# Autodesk Inventor assembly: assem_linact_standalone_newfinger_v2_test
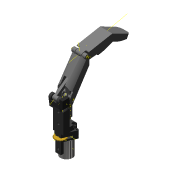
[picture p0: Inventor's stored thumbnail of the model, 180x180]
Saved by Autodesk Inventor 2014 (Build 180170000, 170)
## iProperties
Created: 2015-05-04
Part Number: assem_linact_standalone_newfinger_v2_test
Document SubType Name: Assembly
Designer: Martin
Author: Martin
## Documents named in this file (18)
- C:\Users\Martin\Dropbox\biohand-mec\biohand_v1\fingers\middle\assem_finger_middle.iam
- C:\Users\Martin\Dropbox\biohand-mec\biohand_v1\fingers\index\linact_knuckle_v2.ipt
- C:\Users\Martin\Dropbox\biohand-mec\biohand_v1\fingers\index\assem_linact_rod_v3.iam
- C:\Users\Martin\Dropbox\biohand-mec\biohand_v1\fingers\middle\finger_proximal_v2.ipt
- C:\Users\Martin\Dropbox\biohand-mec\biohand_v1\fingers\index\finger_clevislink.ipt
- C:\Users\Martin\Dropbox\biohand-mec\biohand_v1\misc\servo_square_pot.ipt
- C:\Users\Martin\Dropbox\biohand-mec\biohand_v1\fingers\middle\finger_link_v2.ipt
- C:\Users\Martin\Dropbox\biohand-mec\biohand_v1\fingers\middle\finger_distal.ipt
- C:\Users\Martin\Dropbox\biohand-mec\biohand_v1\misc\bearing_10_4_3.ipt
- C:\Users\Martin\Dropbox\biohand-mec\biohand_v1\misc\m3_25_screw.ipt
- C:\Users\Martin\Dropbox\biohand-mec\biohand_v1\misc\m3_nut.ipt
- C:\Users\Martin\Dropbox\biohand-mec\biohand_v1\misc\servo_gear_2.ipt
- C:\Users\Martin\Dropbox\biohand-mec\biohand_v1\fingers\index\linact_top.ipt
- C:\Users\Martin\Dropbox\biohand-mec\biohand_v1\fingers\index\linact_base.ipt
- C:\Users\Martin\Dropbox\biohand-mec\biohand_v1\misc\m2_8_screw.ipt
- C:\Users\Martin\Dropbox\biohand-mec\biohand_v1\misc\motor_servo.ipt
- C:\Users\Martin\Dropbox\biohand-mec\biohand_v1\misc\m2_4_screw.ipt
- C:\Users\Martin\Dropbox\biohand-mec\biohand_v1\misc\servo_gear_1.ipt
## Components (23 placed, 17 different names)
1. linact_knuckle_v2:1 — Mate:1, Mate:2, Insert:1, Insert:3, Insert:4, Insert:6, Mate:6, Mate:7, Mate:8, Insert:12
2. assem_linact_rod_v3:1 [sub-assembly] — Mate:1, Mate:2, Insert:2
3. finger_proximal_v2:1 — Insert:1, Mate:3, Insert:5, Angle:2, Insert:9, Insert:14, Insert:15, Insert:16, Insert:17, Insert:18, Insert:19
4. finger_clevislink:1 — Insert:2, Mate:3
5. servo_square_pot:1 — Insert:3, Angle:1
6. finger_link_v2:1 — Insert:4, Mate:4, Insert:10
7. finger_distal:1 — Insert:5, Mate:4, Insert:9
8. bearing_10_4_3:1 — Insert:6, Insert:8
9. m3_25_screw:1 — Insert:7
10. m3_nut:1 — Mate:5, Insert:8
11. servo_gear_2:1 — Mate:5, Insert:7
12. linact_top:1 — Mate:6, Mate:7, Mate:8, Mate:9, Mate:10, Mate:11, Insert:13
13. linact_base:1 — Mate:9, Mate:10, Mate:11, Insert:11
14. m2_8_screw:1 — Insert:10
15. motor_servo:1 — Insert:11, Angle:3
16. m2_4_screw:1 — Insert:12
17. servo_gear_1:1 — Insert:13
18. m2_8_screw:2 — Insert:14
19. m2_8_screw:3 — Insert:15
20. m2_8_screw:4 — Insert:18
21. m2_8_screw:5 — Insert:16
22. m2_8_screw:6 — Insert:17
23. m2_8_screw:7 — Insert:19
## Relationships (33: Insert 19, Mate 11, Angle 3)
- Mate:1: linact_knuckle_v2:1 ↔ assem_linact_rod_v3:1
- Mate:2 (0.2 mm): linact_knuckle_v2:1 ↔ assem_linact_rod_v3:1
- Insert:1 (0.75 mm): linact_knuckle_v2:1 ↔ finger_proximal_v2:1
- Insert:2 (0.25 mm): assem_linact_rod_v3:1 ↔ finger_clevislink:1
- Mate:3: finger_proximal_v2:1 ↔ finger_clevislink:1
- Insert:3: linact_knuckle_v2:1 ↔ servo_square_pot:1
- Angle:1 (180 deg): servo_square_pot:1
- Insert:4 (0.5 mm): linact_knuckle_v2:1 ↔ finger_link_v2:1
- Insert:5 (0.5 mm): finger_proximal_v2:1 ↔ finger_distal:1
- Mate:4: finger_link_v2:1 ↔ finger_distal:1
- Insert:6: linact_knuckle_v2:1 ↔ bearing_10_4_3:1
- Mate:5: m3_nut:1 ↔ servo_gear_2:1
- Insert:7: m3_25_screw:1 ↔ servo_gear_2:1
- Insert:8: bearing_10_4_3:1 ↔ m3_nut:1
- Angle:2 (180 deg): finger_proximal_v2:1
- Mate:6: linact_knuckle_v2:1 ↔ linact_top:1
- Mate:7: linact_knuckle_v2:1 ↔ linact_top:1
- Mate:8: linact_knuckle_v2:1 ↔ linact_top:1
- Mate:9: linact_top:1 ↔ linact_base:1
- Mate:10: linact_top:1 ↔ linact_base:1
- Mate:11: linact_top:1 ↔ linact_base:1
- Insert:9 (0.5 mm): finger_proximal_v2:1 ↔ finger_distal:1
- Insert:10: finger_link_v2:1 ↔ m2_8_screw:1
- Insert:11: linact_base:1 ↔ motor_servo:1
- Angle:3 (0 deg): motor_servo:1
- Insert:12: linact_knuckle_v2:1 ↔ m2_4_screw:1
- Insert:13 (0.3 mm): linact_top:1 ↔ servo_gear_1:1
- Insert:14: finger_proximal_v2:1 ↔ m2_8_screw:2
- Insert:15: finger_proximal_v2:1 ↔ m2_8_screw:3
- Insert:16: finger_proximal_v2:1 ↔ m2_8_screw:5
- Insert:17: finger_proximal_v2:1 ↔ m2_8_screw:6
- Insert:18: finger_proximal_v2:1 ↔ m2_8_screw:4
- Insert:19: finger_proximal_v2:1 ↔ m2_8_screw:7
